# Autodesk Inventor assembly: Bumper
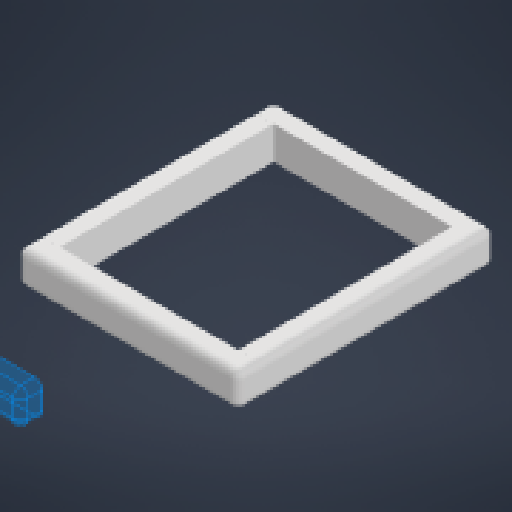
[picture p0: Inventor's stored thumbnail of the model, 512x512]
Saved by Autodesk Inventor 2023 (Build 270158000, 158)
## iProperties
Created: 2023-01-12
Part Number: Bumper
Document SubType Name: Assembly
Designer: Terrence
Author: Terrence
## Documents named in this file (3)
- C:\Users\Terrence\Documents\FRC Long\Bumper\Bumper.iam
- C:\Users\Terrence\Documents\FRC Long\Bumper\Solid1.ipt
- C:\Users\Terrence\Documents\FRC Long\Bumper\Solid2.ipt
## Components (4 placed, 2 different names)
1. Solid1:1 — Flush:3, Flush:4
2. Solid2:1 — Mate:1, Flush:1, Flush:2
3. Solid1:2 — Mate:1, Flush:1, Flush:2, Mate:2
4. Solid2:2 — Mate:2, Flush:3, Flush:4
## Relationships (6: Flush 4, Mate 2)
- Mate:1: Solid2:1 ↔ Solid1:2
- Flush:1: Solid2:1 ↔ Solid1:2
- Flush:2: Solid2:1 ↔ Solid1:2
- Mate:2: Solid1:2 ↔ Solid2:2
- Flush:3: Solid1:1 ↔ Solid2:2
- Flush:4: Solid1:1 ↔ Solid2:2
